# Autodesk Inventor assembly: 50cal
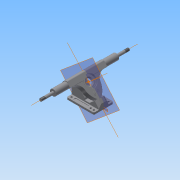
[picture p0: Inventor's stored thumbnail of the model, 180x180]
Saved by Autodesk Inventor 2015 (Build 190159000, 159)
## iProperties
Created: 2014-11-13
Part Number: 50cal
Document SubType Name: Assembly
Designer: brent
Author: brent
## Documents named in this file (3)
- C:\Users\brent\Documents\electric-longboard\brent2\50cal.iam
- C:\Users\brent\Documents\electric-longboard\brent2\50cal_baseplate.ipt
- C:\Users\brent\Documents\electric-longboard\brent2\50cal_hanger.ipt
## Components (2 placed, 2 different names)
1. 50cal_baseplate:1 — Mate:1, Mate:2, Mate:3, Mate:6
2. 50cal_hanger:1 — Mate:1, Mate:2, Mate:5, Mate:6
## Relationships (5: Mate 5)
- Mate:1: 50cal_baseplate:1 ↔ 50cal_hanger:1
- Mate:2: 50cal_baseplate:1 ↔ 50cal_hanger:1
- Mate:3: 50cal_baseplate:1
- Mate:5: 50cal_hanger:1
- Mate:6: 50cal_baseplate:1 ↔ 50cal_hanger:1
